# Autodesk Inventor assembly: Assembly1
(part 3 of 3)
- Mate:657: Loslagertopf:1 ↔ Schutzpuffer:1
## Named parameters: d42_d40 = 0 mm, d43_d41 = 0 mm, d44_d40 = 0 mm, d45_d41 = 0 mm, d148_d145 = 0 mm, d149_d146 = 0 mm, d150_d147 = 0 deg, d151_d145 = 0 mm, d152_d146 = 0 mm, d153_d147 = 0 deg, d154_d145 = 0 mm, d155_d146 = 0 mm, d156_d147 = 0 deg, d157_d145 = 0 mm, d158_d146 = 0 mm, d159_d147 = 0 deg, d206_d203 = 0 mm, d207_d205 = 0 mm, d212_d206_d203 = 0 mm, d213_d207_d205 = 0 mm, d214_d206_d203 = 0 mm, d215_d207_d205 = 0 mm, d218_d212_d206_d203 = 0 mm, d219_d213_d207_d205 = 0 mm, d220_d214_d206_d203 = 0 mm, d221_d215_d207_d205 = 0 mm, d222_d210_d206_d203 = 0 mm, d223_d211_d207_d205 = 0 mm, d224_d212_d206_d203 = 0 mm, d225_d213_d207_d205 = 0 mm, d226_d214_d206_d203 = 0 mm, d227_d215_d207_d205 = 0 mm, d228_d216_d210_d206_d203 = 0 mm, d229_d217_d211_d207_d205 = 0 mm, d230_d218_d212_d206_d203 = 0 mm, d231_d219_d213_d207_d205 = 0 mm, d232_d220_d214_d206_d203 = 0 mm, d233_d221_d215_d207_d205 = 0 mm, d234_d210_d206_d203 = 0 mm, d235_d211_d207_d205 = 0 mm, d236_d212_d206_d203 = 0 mm, d237_d213_d207_d205 = 0 mm, d238_d214_d206_d203 = 0 mm, d239_d215_d207_d205 = 0 mm, d240_d216_d210_d206_d203 = 0 mm, d241_d217_d211_d207_d205 = 0 mm, d242_d218_d212_d206_d203 = 0 mm, d243_d219_d213_d207_d205 = 0 mm, d244_d220_d214_d206_d203 = 0 mm, d245_d221_d215_d207_d205 = 0 mm, d287_d285 = 0 mm, d288_d286 = 0 mm, d289_d285 = 0 mm, d290_d286 = 0 mm, d291_d285 = 0 mm, d292_d286 = 0 mm, d301_d285 = 0 mm, d302_d286 = 0 mm, d303_d287_d285 = 0 mm, d304_d288_d286 = 0 mm, d305_d289_d285 = 0 mm, d306_d290_d286 = 0 mm, d307_d291_d285 = 0 mm, d308_d292_d286 = 0 mm, d317_d301_d285 = 0 mm, d318_d302_d286 = 0 mm, d319_d305_d289_d285 = 0 mm, d320_d306_d290_d286 = 0 mm, d321_d307_d291_d285 = 0 mm, d322_d308_d292_d286 = 0 mm, d330_d317_d301_d285 = 0 mm, d331_d318_d302_d286 = 0 mm, d338_d330_d317_d301_d285 = 0 mm, d339_d331_d318_d302_d286 = 0 mm, d340_d330_d317_d301_d285 = 0 mm, d341_d331_d318_d302_d286 = 0 mm, d342_d338_d330_d317_d301_d285 = 0 mm, d343_d339_d331_d318_d302_d286 = 0 mm, d344_d340_d330_d317_d301_d285 = 0 mm, d345_d341_d331_d318_d302_d286 = 0 mm, d346_d338_d330_d317_d301_d285 = 0 mm, d347_d339_d331_d318_d302_d286 = 0 mm, d348_d340_d330_d317_d301_d285 = 0 mm, d349_d341_d331_d318_d302_d286 = 0 mm, d350_d338_d330_d317_d301_d285 = 0 mm, d351_d339_d331_d318_d302_d286 = 0 mm, d352_d340_d330_d317_d301_d285 = 0 mm, d353_d341_d331_d318_d302_d286 = 0 mm, d356_d340_d330_d317_d301_d285 = 0 mm, d357_d341_d331_d318_d302_d286 = 0 mm, d388_d338_d330_d317_d301_d285 = 0 mm, d389_d339_d331_d318_d302_d286 = 0 mm, d390_d338_d330_d317_d301_d285 = 0 mm, d391_d339_d331_d318_d302_d286 = 0 mm, d392_d388_d338_d330_d317_d301_d285 = 0 mm, d393_d389_d339_d331_d318_d302_d286 = 0 mm, d394_d390_d338_d330_d317_d301_d285 = 0 mm, d395_d391_d339_d331_d318_d302_d286 = 0 mm, d396_d388_d338_d330_d317_d301_d285 = 0 mm, d397_d389_d339_d331_d318_d302_d286 = 0 mm, d398_d390_d338_d330_d317_d301_d285 = 0 mm, d399_d391_d339_d331_d318_d302_d286 = 0 mm, d414_d394_d390_d338_d330_d317_d301_d285 = 0 mm, d415_d395_d391_d339_d331_d318_d302_d286 = 0 mm, d416_d414_d394_d390_d338_d330_d317_d301_d285 = 0 mm, d417_d415_d395_d391_d339_d331_d318_d302_d286 = 0 mm, d418_d414_d394_d390_d338_d330_d317_d301_d285 = 0 mm, d419_d415_d395_d391_d339_d331_d318_d302_d286 = 0 mm, d422_d414_d394_d390_d338_d330_d317_d301_d285 = 0 mm, d423_d415_d395_d391_d339_d331_d318_d302_d286 = 0 mm, d426_d414_d394_d390_d338_d330_d317_d301_d285 = 0 mm, d427_d415_d395_d391_d339_d331_d318_d302_d286 = 0 mm, d438_d414_d394_d390_d338_d330_d317_d301_d285 = 0 mm, d439_d415_d395_d391_d339_d331_d318_d302_d286 = 0 mm, d537_d321_d307_d291_d285 = 0 mm, d538_d322_d308_d292_d286 = 0 mm, d539_d537_d321_d307_d291_d285 = 0 mm, d540_d538_d322_d308_d292_d286 = 0 mm, d541_d537_d321_d307_d291_d285 = 0 mm, d542_d538_d322_d308_d292_d286 = 0 mm, d543_d537_d321_d307_d291_d285 = 0 mm, d544_d538_d322_d308_d292_d286 = 0 mm, d545_d537_d321_d307_d291_d285 = 0 mm, d546_d538_d322_d308_d292_d286 = 0 mm, d547_d537_d321_d307_d291_d285 = 0 mm, d548_d538_d322_d308_d292_d286 = 0 mm, d549_d537_d321_d307_d291_d285 = 0 mm, d550_d538_d322_d308_d292_d286 = 0 mm, d551_d537_d321_d307_d291_d285 = 0 mm, d552_d538_d322_d308_d292_d286 = 0 mm, d568_d551_d537_d321_d307_d291_d285 = 0 mm, d569_d552_d538_d322_d308_d292_d286 = 0 mm, d570_d551_d537_d321_d307_d291_d285 = 0 mm, d571_d552_d538_d322_d308_d292_d286 = 0 mm, d572_d551_d537_d321_d307_d291_d285 = 0 mm, d573_d552_d538_d322_d308_d292_d286 = 0 mm, d574_d551_d537_d321_d307_d291_d285 = 0 mm, d575_d552_d538_d322_d308_d292_d286 = 0 mm, d609_d607 = 0 mm, d610_d608 = 0 mm, d611_d607 = 0 mm, d612_d608 = 0 mm, d613_d609_d607 = 0 mm, d614_d610_d608 = 0 mm, d615_d607 = 0 mm, d616_d608 = 0 mm, d617_d609_d607 = 0 mm, d618_d610_d608 = 0 mm, d736_d537_d321_d307_d291_d285 = 0 mm, d737_d538_d322_d308_d292_d286 = 0 mm, d738_d736_d537_d321_d307_d291_d285 = 0 mm, d739_d737_d538_d322_d308_d292_d286 = 0 mm, d740_d736_d537_d321_d307_d291_d285 = 0 mm, d741_d737_d538_d322_d308_d292_d286 = 0 mm, d742_d736_d537_d321_d307_d291_d285 = 0 mm, d743_d737_d538_d322_d308_d292_d286 = 0 mm
